# Autodesk Inventor assembly: Toughbox Hex Output Shaft
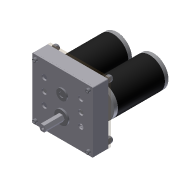
[picture p0: Inventor's stored thumbnail of the model, 180x180]
Saved by Autodesk Inventor 2011 (Build 150239000, 239)
## iProperties
Created: 2012-06-01
Part Number: Toughbox Hex Output Shaft
Document SubType Name: Assembly
Designer: Nemo
Author: Nemo
## Documents named in this file (15)
- H:\Nemo\Documents\Robotics\COTS Parts\Gearboxes\Toughbox Hex Output Shaft.iam
- H:\Nemo\Documents\Robotics\COTS Parts\Gearboxes\Housings\Toughbox Motor Plate.ipt
- H:\Nemo\Documents\Robotics\COTS Parts\Gearboxes\Bearings\Bearing FR6zz.ipt
- H:\Nemo\Documents\Robotics\COTS Parts\Gearboxes\Shafts\Toughbox Small Hex Shaft.ipt
- H:\Nemo\Documents\Robotics\COTS Parts\Gearboxes\Gears\Gear 20dp 375hex 50T.ipt
- H:\Nemo\Documents\Robotics\COTS Parts\Gearboxes\Gears\Gear 20dp 375hex 14T.ipt
- H:\Nemo\Documents\Robotics\COTS Parts\Gearboxes\Shafts\Toughbox Hex Output Shaft.ipt
- H:\Nemo\Documents\Robotics\COTS Parts\Gearboxes\Gears\Gear 20dp 500hex 50T.ipt
- H:\Nemo\Documents\Robotics\COTS Parts\Gearboxes\Housings\Toughbox Enclosure.ipt
- H:\Nemo\Documents\Robotics\COTS Parts\Gearboxes\Housings\Toughbox Shaft Plate.ipt
- H:\Nemo\Documents\Robotics\COTS Parts\Gearboxes\Bearings\Bearing FR8zz-hex.ipt
- H:\Nemo\Documents\Robotics\COTS Parts\Motors\CIM Motor 14T.iam
- H:\Nemo\Documents\Robotics\COTS Parts\Fasteners\10-32 SHCS x1750.ipt
- H:\Nemo\Documents\Robotics\COTS Parts\Fasteners\14-20 locknut.ipt
- H:\Nemo\Documents\Robotics\COTS Parts\Fasteners\10-32 SHCS x625.ipt
## Components (26 placed, 14 different names)
1. Toughbox Motor Plate:1 — Insert:1, Insert:2, Mate:6, Flush:2, Flush:3, Mate:7, Mate:8, Insert:8, Mate:10, Insert:9, Mate:11, Insert:14, Insert:15, Insert:16, Insert:17, Insert:23, Insert:24, Insert:25
2. Bearing FR6zz:1 — Insert:1, Insert:3, Mate:2
3. Bearing FR6zz:2 — Insert:2, Insert:4
4. Toughbox Cluster Shaft 375hex:1 — Insert:3, Mate:1, Angle:1, Mate:3
5. Gear 20dp 375hex 50T:1 — Mate:1, Angle:1, Mate:2, Mate:4
6. Gear 14T 20dp 375hex:1 — Mate:3, Mate:4
7. Toughbox Hex Output Shaft:1 — Insert:4, Mate:5, Angle:2, Flush:1, Angle:3
8. Gear 50T 20dp 500hex:1 — Mate:5, Angle:2, Flush:1
9. Toughbox Enclosure:1 — Mate:6, Flush:2, Flush:3, Mate:9
10. Toughbox Shaft Plate:1 — Mate:7, Mate:8, Insert:6, Insert:7, Mate:9, Insert:18, Insert:19, Insert:20, Insert:21
11. Bearing FR6zz:3 — Insert:7
12. Bearing FR8zz-hex:1 — Insert:6, Angle:3
13. CIM Motor 14T:1 [sub-assembly] — Insert:9, Mate:11, Insert:22
14. CIM Motor 14T:2 [sub-assembly] — Insert:8, Mate:10
15. 10-32 SHCS x1750:1 — Insert:20
16. 10-32 SHCS x1750:2 — Insert:21
17. 10-32 SHCS x1750:3 — Insert:19
18. 10-32 SHCS x1750:4 — Insert:18
19. 14-20 locknut:1 — Insert:17
20. 14-20 locknut:2 — Insert:16
21. 14-20 locknut:3 — Insert:15
22. 14-20 locknut:4 — Insert:14
23. 10-32 SHCS x625:1 — Insert:25
24. 10-32 SHCS x625:2 — Insert:24
25. 10-32 SHCS x625:3 — Insert:23
26. 10-32 SHCS x625:4 — Insert:22
## Relationships (37: Insert 20, Mate 11, Angle 3, Flush 3)
- Insert:1: Toughbox Motor Plate:1 ↔ Bearing FR6zz:1
- Insert:2: Toughbox Motor Plate:1 ↔ Bearing FR6zz:2
- Insert:3: Bearing FR6zz:1 ↔ Toughbox Cluster Shaft 375hex:1
- Mate:1: Toughbox Cluster Shaft 375hex:1 ↔ Gear 20dp 375hex 50T:1
- Angle:1 (0 deg): Toughbox Cluster Shaft 375hex:1 ↔ Gear 20dp 375hex 50T:1
- Mate:2: Bearing FR6zz:1 ↔ Gear 20dp 375hex 50T:1
- Mate:3: Toughbox Cluster Shaft 375hex:1 ↔ Gear 14T 20dp 375hex:1
- Mate:4: Gear 20dp 375hex 50T:1 ↔ Gear 14T 20dp 375hex:1
- Insert:4: Bearing FR6zz:2 ↔ Toughbox Hex Output Shaft:1
- Mate:5: Toughbox Hex Output Shaft:1 ↔ Gear 50T 20dp 500hex:1
- Angle:2 (0 deg): Toughbox Hex Output Shaft:1 ↔ Gear 50T 20dp 500hex:1
- Flush:1: Toughbox Hex Output Shaft:1 ↔ Gear 50T 20dp 500hex:1
- Mate:6: Toughbox Motor Plate:1 ↔ Toughbox Enclosure:1
- Flush:2: Toughbox Motor Plate:1 ↔ Toughbox Enclosure:1
- Flush:3: Toughbox Motor Plate:1 ↔ Toughbox Enclosure:1
- Mate:7: Toughbox Motor Plate:1 ↔ Toughbox Shaft Plate:1
- Mate:8: Toughbox Motor Plate:1 ↔ Toughbox Shaft Plate:1
- Insert:6: Toughbox Shaft Plate:1 ↔ Bearing FR8zz-hex:1
- Insert:7: Toughbox Shaft Plate:1 ↔ Bearing FR6zz:3
- Angle:3 (0 deg): Toughbox Hex Output Shaft:1 ↔ Bearing FR8zz-hex:1
- Mate:9: Toughbox Enclosure:1 ↔ Toughbox Shaft Plate:1
- Insert:8: Toughbox Motor Plate:1 ↔ CIM Motor 14T:2
- Mate:10: Toughbox Motor Plate:1 ↔ CIM Motor 14T:2
- Insert:9: Toughbox Motor Plate:1 ↔ CIM Motor 14T:1
- Mate:11: Toughbox Motor Plate:1 ↔ CIM Motor 14T:1
- Insert:14: Toughbox Motor Plate:1 ↔ 14-20 locknut:4
- Insert:15: Toughbox Motor Plate:1 ↔ 14-20 locknut:3
- Insert:16: Toughbox Motor Plate:1 ↔ 14-20 locknut:2
- Insert:17: Toughbox Motor Plate:1 ↔ 14-20 locknut:1
- Insert:18: Toughbox Shaft Plate:1 ↔ 10-32 SHCS x1750:4
- Insert:19: Toughbox Shaft Plate:1 ↔ 10-32 SHCS x1750:3
- Insert:20: Toughbox Shaft Plate:1 ↔ 10-32 SHCS x1750:1
- Insert:21: Toughbox Shaft Plate:1 ↔ 10-32 SHCS x1750:2
- Insert:22: CIM Motor 14T:1 ↔ 10-32 SHCS x625:4
- Insert:23: Toughbox Motor Plate:1 ↔ 10-32 SHCS x625:3
- Insert:24: Toughbox Motor Plate:1 ↔ 10-32 SHCS x625:2
- Insert:25: Toughbox Motor Plate:1 ↔ 10-32 SHCS x625:1
